# Autodesk Inventor assembly: TapaEje
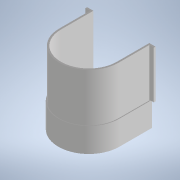
[picture p0: Inventor's stored thumbnail of the model, 180x180]
Saved by Autodesk Inventor 2020 (Build 240168000, 168)
## iProperties
Created: 2019-11-12
Part Number: TapaEje
Document SubType Name: Assembly
Designer: Usuario
Author: Usuario
## Documents named in this file (3)
- G:\Mi unidad\UTEC\Proyectos\Flor de Lana\Diseño 20191016\TapaEje.iam
- G:\Mi unidad\UTEC\Proyectos\Flor de Lana\Diseño 20191016\TapaEje1.ipt
- G:\Mi unidad\UTEC\Proyectos\Flor de Lana\Diseño 20191016\TapaEje2.ipt
## Components (2 placed, 2 different names)
1. TapaEje1:1 — De rotación:1
2. TapaEje2:1 — De rotación:1
## Relationships (1: RevoluteJoint 1)
- De rotación:1 [RevoluteJoint]: TapaEje1:1 ↔ TapaEje2:1
